# Autodesk Inventor assembly: EnsamblajeCasa
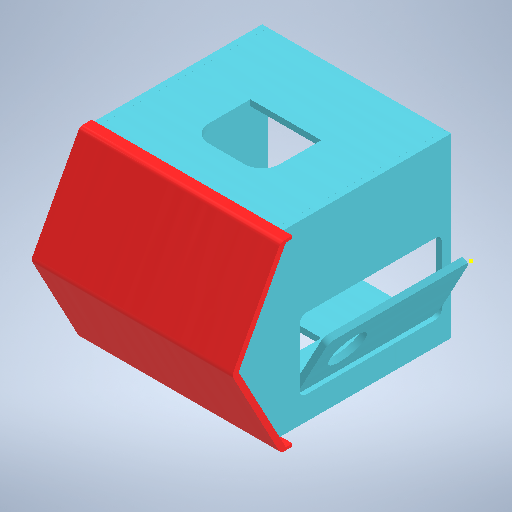
[picture p0: Inventor's stored thumbnail of the model, 512x512]
Saved by Autodesk Inventor 2025.2 (Build 292293000, 293)
## iProperties
Created: 2025-01-19
Part Number: EnsamblajeCasa
Document SubType Name: Assembly
Designer: usuario
Author: usuario
## Documents named in this file (6)
- C:\Users\usuario\Desktop\ModeladosAPM\CASA\EnsamblajeCasa.iam
- C:\Users\usuario\Desktop\ModeladosAPM\CASA\ParedDelanteraCasa.ipt
- C:\Users\usuario\Desktop\ModeladosAPM\CASA\ParedLateralCasa.ipt
- C:\Users\usuario\Desktop\ModeladosAPM\CASA\ParedTraseraCasa.ipt
- C:\Users\usuario\Desktop\ModeladosAPM\CASA\Puerta.ipt
- C:\Users\usuario\Desktop\ModeladosAPM\CASA\TechoCasa.ipt
## Components (6 placed, 5 different names)
1. ParedDelanteraCasa:1 — Coincidencia:1, Coincidencia:2, Coincidencia:5, Coincidencia:6, Coincidencia:7, Coincidencia:8, Coincidencia:9, Coincidencia:10, Coincidencia:11
2. ParedLateralCasa:1 — Coincidencia:5, Coincidencia:6
3. ParedTraseraCasa:1 — Coincidencia:3, Coincidencia:4, Nivelación:1
4. Puerta:1 — Coincidencia:8, Coincidencia:9
5. TechoCasa:1 — Coincidencia:10, Coincidencia:11
6. ParedLateralCasa:2 — Coincidencia:1, Coincidencia:2, Coincidencia:3, Coincidencia:4, Nivelación:1, Coincidencia:7
## Relationships (12: Mate 11, Flush 1)
- Coincidencia:1 [Mate]: ParedDelanteraCasa:1 ↔ ParedLateralCasa:2
- Coincidencia:2 [Mate]: ParedDelanteraCasa:1 ↔ ParedLateralCasa:2
- Coincidencia:3 [Mate]: ParedTraseraCasa:1 ↔ ParedLateralCasa:2
- Coincidencia:4 [Mate]: ParedTraseraCasa:1 ↔ ParedLateralCasa:2
- Coincidencia:5 [Mate]: ParedDelanteraCasa:1 ↔ ParedLateralCasa:1
- Coincidencia:6 [Mate]: ParedDelanteraCasa:1 ↔ ParedLateralCasa:1
- Nivelación:1 [Flush]: ParedTraseraCasa:1 ↔ ParedLateralCasa:2
- Coincidencia:7 [Mate]: ParedDelanteraCasa:1 ↔ ParedLateralCasa:2
- Coincidencia:8 [Mate]: ParedDelanteraCasa:1 ↔ Puerta:1
- Coincidencia:9 [Mate]: ParedDelanteraCasa:1 ↔ Puerta:1
- Coincidencia:10 [Mate]: ParedDelanteraCasa:1 ↔ TechoCasa:1
- Coincidencia:11 [Mate]: ParedDelanteraCasa:1 ↔ TechoCasa:1
